# Autodesk Inventor assembly: 200-60-DIFFERENTIAL-CONNECTOR-02
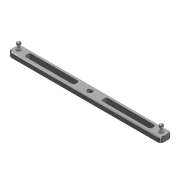
[picture p0: Inventor's stored thumbnail of the model, 180x180]
Saved by Autodesk Inventor 2018.2 (Build 222227000, 227)
## iProperties
Manager: feesmrt
Company: FRANC0R
Created: 2017-12-19
Part Number: 200-60-DIFFERENTIAL-CONNECTOR-02
Project: Rescue Robot
Cost Center: -
Material: Generisch
Document SubType Name: Assembly
Designer: feesmrt
Engineer: feesmrt
Authority: feesmrt
Description: Differential Connector Arm
Stock Number: 200-60-DIFFERENTIAL-CONNECTOR-02
Subject: Rescue Robot
Author: feesmrt
Revision Number: 1
Title: Differential Connector Arm
## Documents named in this file (4)
- D:\Programmierung\FRANC0R\CAD\02-Rocker-Bogie-Robot\200-ROCKER-BOGIE\200-60-DIFFERENTIAL\200-60-DIFFERENTIAL-CONNECTOR-02.iam
- D:\Programmierung\FRANC0R\CAD\02-Rocker-Bogie-Robot\200-ROCKER-BOGIE\200-60-DIFFERENTIAL\200-60-DIFFERENTIAL-CONNECTOR-01.ipt
- D:\Programmierung\FRANC0R\CAD\02-Rocker-Bogie-Robot\900-COMPONENTS\900-70-ANGLE-JOINTS\900-70-ANGLE-JOINTS-DIN71802-M6-2.ipt
- D:\Programmierung\FRANC0R\CAD\02-Rocker-Bogie-Robot\900-COMPONENTS\900-80-WASHERS\900-80-WASHERS-ISO8738-6.ipt
## Components (7 placed, 3 different names)
1. 200-60-DIFFERENTIAL-CONNECTOR-01:1 — Passend:5, Passend:6, Winkel:1, Passend:11, Passend:12, Winkel:2
2. 900-70-ANGLE-JOINTS-DIN71802-M6-2:1 — Passend:1, Passend:2, Passend:3, Passend:5, Winkel:1
3. 900-70-ANGLE-JOINTS-DIN71802-M6-2:2 — Passend:7, Passend:8, Passend:9, Passend:11, Winkel:2
4. 900-80-WASHERS-ISO8738-6:1 — Passend:1, Passend:3, Passend:4
5. 900-80-WASHERS-ISO8738-6:2 — Passend:2, Passend:4, Passend:6
6. 900-80-WASHERS-ISO8738-6:3 — Passend:8, Passend:10, Passend:12
7. 900-80-WASHERS-ISO8738-6:4 — Passend:7, Passend:9, Passend:10
## Relationships (14: Mate 12, Angle 2)
- Passend:1 [Mate]: 900-70-ANGLE-JOINTS-DIN71802-M6-2:1 ↔ 900-80-WASHERS-ISO8738-6:1
- Passend:2 [Mate]: 900-70-ANGLE-JOINTS-DIN71802-M6-2:1 ↔ 900-80-WASHERS-ISO8738-6:2
- Passend:3 [Mate]: 900-70-ANGLE-JOINTS-DIN71802-M6-2:1 ↔ 900-80-WASHERS-ISO8738-6:1
- Passend:4 [Mate]: 900-80-WASHERS-ISO8738-6:1 ↔ 900-80-WASHERS-ISO8738-6:2
- Passend:5 [Mate]: 200-60-DIFFERENTIAL-CONNECTOR-01:1 ↔ 900-70-ANGLE-JOINTS-DIN71802-M6-2:1
- Passend:6 [Mate]: 200-60-DIFFERENTIAL-CONNECTOR-01:1 ↔ 900-80-WASHERS-ISO8738-6:2
- Winkel:1 [Angle] (0 deg): 200-60-DIFFERENTIAL-CONNECTOR-01:1 ↔ 900-70-ANGLE-JOINTS-DIN71802-M6-2:1
- Passend:7 [Mate]: 900-70-ANGLE-JOINTS-DIN71802-M6-2:2 ↔ 900-80-WASHERS-ISO8738-6:4
- Passend:8 [Mate]: 900-70-ANGLE-JOINTS-DIN71802-M6-2:2 ↔ 900-80-WASHERS-ISO8738-6:3
- Passend:9 [Mate]: 900-70-ANGLE-JOINTS-DIN71802-M6-2:2 ↔ 900-80-WASHERS-ISO8738-6:4
- Passend:10 [Mate]: 900-80-WASHERS-ISO8738-6:3 ↔ 900-80-WASHERS-ISO8738-6:4
- Passend:11 [Mate]: 200-60-DIFFERENTIAL-CONNECTOR-01:1 ↔ 900-70-ANGLE-JOINTS-DIN71802-M6-2:2
- Passend:12 [Mate]: 200-60-DIFFERENTIAL-CONNECTOR-01:1 ↔ 900-80-WASHERS-ISO8738-6:3
- Winkel:2 [Angle] (0 deg): 200-60-DIFFERENTIAL-CONNECTOR-01:1 ↔ 900-70-ANGLE-JOINTS-DIN71802-M6-2:2
